# Autodesk Inventor assembly: ASM Printing Head
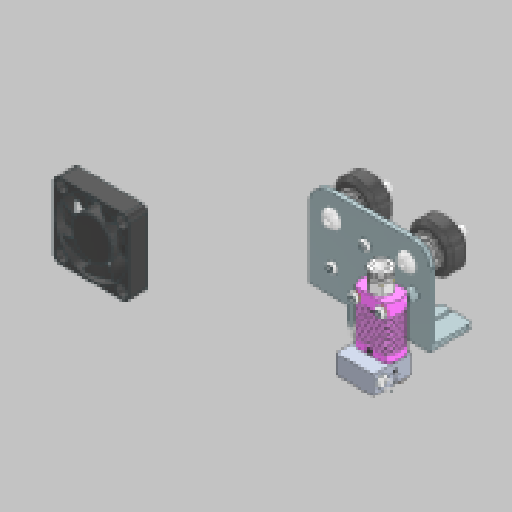
[picture p0: Inventor's stored thumbnail of the model, 512x512]
Saved by Autodesk Inventor 2025.4 (Build 294407000, 407)
## iProperties
Created: 2026-03-02
Part Number: ASM Printing Head
Document SubType Name: Assembly
Designer: Inema
Author: Inema
Revision Number: ANY
## Documents named in this file (8)
- C:\Users\Inema\OneDrive\GitHub\Ender-3\Ender-3 Mechanical\Modificada\Extrusor Original\ASM Printing Head.iam
- C:\Users\Inema\OneDrive\GitHub\Ender-3\Ender-3 Mechanical\Modificada\Extrusor Original\E plate.ipt
- C:\Users\Inema\OneDrive\GitHub\Ender-3\Ender-3 Mechanical\Modificada\Extrusor Original\Nozzle fan.ipt
- C:\Users\Inema\OneDrive\GitHub\Ender-3\Ender-3 Mechanical\Modificada\Extrusor Original\ASM Heating Unit.iam
- C:\Users\Inema\OneDrive\GitHub\Ender-3\Ender-3 Mechanical\Modificada\Extrusor Original\ASM Roller X-Axis.iam
- C:\Users\Inema\OneDrive\GitHub\Ender-3\Ender-3 Mechanical\Modificada\Extrusor Original\ASM Eccentrical Roller X-Axis.iam
- C:\Users\Inema\OneDrive\GitHub\Ender-3\Ender-3 Mechanical\Modificada\Extrusor Original\M3X6Pan Head Screw.ipt
- C:\Users\Inema\OneDrive\GitHub\Ender-3\Ender-3 Mechanical\Modificada\direct_drive_extruder_bracket_v1.3\direct_drive_extruder_bracket_v1.3\direct_drive_extruder_bracket_v1.3.ipt
## Components (9 placed, 9 different names)
1. E plate_168 — Coincidencia:1
2. Nozzle fan_172
3. ASM Heating Unit_173 [sub-assembly]
4. ASM Roller X-Axis_174 [sub-assembly] — Coincidencia:2
5. ASM Roller X-Axis_175 [sub-assembly] — Coincidencia:3
6. ASM Eccentrical Roller X-Axis_176 [sub-assembly]
7. M3X6Pan Head Screw_182
8. M3X6Pan Head Screw_183
9. direct_drive_extruder_bracket_v1.3:1 — Coincidencia:1, Coincidencia:2, Coincidencia:3
## Relationships (3: Mate 3)
- Coincidencia:1 [Mate]: E plate_168 ↔ direct_drive_extruder_bracket_v1.3:1
- Coincidencia:2 [Mate]: ASM Roller X-Axis_174 ↔ direct_drive_extruder_bracket_v1.3:1
- Coincidencia:3 [Mate]: ASM Roller X-Axis_175 ↔ direct_drive_extruder_bracket_v1.3:1
